# Autodesk Inventor assembly: Assembly Rotation mechanism
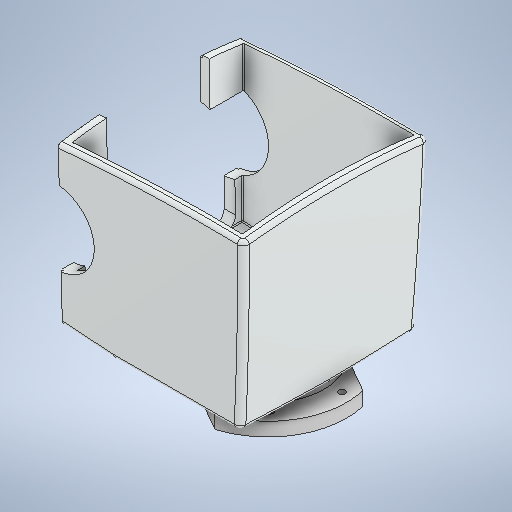
[picture p0: Inventor's stored thumbnail of the model, 512x512]
Saved by Autodesk Inventor 2025.2 (Build 292293000, 293)
## iProperties
Created: 2025-01-03
Part Number: Assembly Rotation mechanism
Document SubType Name: Assembly
Designer: marco.benkert
Author: marco.benkert
## Documents named in this file (6)
- O:\Inventor SanaBike Series\SanaBike 500 Modifield\Rotation Mechanism\Assembly Rotation mechanism.iam
- O:\Inventor SanaBike Series\SanaBike 500 Modifield\Rotation Mechanism\27-30-400 Bearing, Housing Measuring Head.ipt
- O:\Inventor SanaBike Series\SanaBike 500 Modifield\Rotation Mechanism\35-30-xxx Plain Bearing Socket.ipt
- O:\Inventor SanaBike Series\SanaBike 500 Modifield\Rotation Mechanism\25-30-100  Handlebar Cover.ipt
- O:\Inventor SanaBike Series\SanaBike 500 Modifield\Rotation Mechanism\Passscheibe 40x50x1,2 - DIN 988 (ArtNr. 42-03-007)\Passscheibe 40x50x1,2 - DIN 988 (ArtNr. 42-03-007).ipt
- O:\Inventor SanaBike Series\SanaBike 500 Modifield\Rotation Mechanism\Linsenflanschkopf (ecosyn-fix) M4x8 BN4825 (40-08-015)\Linsenflanschkopf (ecosyn-fix) M4x8 BN4825 (40-08-015).ipt
## Components (8 placed, 5 different names)
1. 27-30-400 Bearing, Housing Measuring Head:1 — Mate:6, Flush:1, Mate:7, Mate:10, Flush:2
2. 35-30-xxx Plain Bearing Socket:1 — Rotational:1, Mate:6, Flush:1
3. 25-30-100  Handlebar Cover:1 — Rotational:1, Mate:8, Mate:9, Mate:11, Mate:12, Mate:14, Mate:16
4. Passscheibe 40x50x1,2 - DIN 988 (ArtNr. 42-03-007):1 — Mate:7, Mate:8, Mate:13, Mate:15, Mate:17
5. Linsenflanschkopf (ecosyn-fix) M4x8 BN4825 (40-08-015):1 — Mate:12, Mate:13
6. Linsenflanschkopf (ecosyn-fix) M4x8 BN4825 (40-08-015):2 — Mate:16, Mate:17
7. Linsenflanschkopf (ecosyn-fix) M4x8 BN4825 (40-08-015):3 — Mate:14, Mate:15
8. Passscheibe 40x50x1,2 - DIN 988 (ArtNr. 42-03-007):2 — Mate:9, Mate:10
## Relationships (15: Mate 12, Flush 2, RevoluteJoint 1)
- Rotational:1 [RevoluteJoint]: 35-30-xxx Plain Bearing Socket:1 ↔ 25-30-100  Handlebar Cover:1
- Mate:6: 27-30-400 Bearing, Housing Measuring Head:1 ↔ 35-30-xxx Plain Bearing Socket:1
- Flush:1: 27-30-400 Bearing, Housing Measuring Head:1 ↔ 35-30-xxx Plain Bearing Socket:1
- Mate:7: 27-30-400 Bearing, Housing Measuring Head:1 ↔ Passscheibe 40x50x1,2 - DIN 988 (ArtNr. 42-03-007):1
- Mate:8: 25-30-100  Handlebar Cover:1 ↔ Passscheibe 40x50x1,2 - DIN 988 (ArtNr. 42-03-007):1
- Mate:9: 25-30-100  Handlebar Cover:1 ↔ Passscheibe 40x50x1,2 - DIN 988 (ArtNr. 42-03-007):2
- Mate:10: 27-30-400 Bearing, Housing Measuring Head:1 ↔ Passscheibe 40x50x1,2 - DIN 988 (ArtNr. 42-03-007):2
- Flush:2: 27-30-400 Bearing, Housing Measuring Head:1
- Mate:11: 25-30-100  Handlebar Cover:1
- Mate:12: 25-30-100  Handlebar Cover:1 ↔ Linsenflanschkopf (ecosyn-fix) M4x8 BN4825 (40-08-015):1
- Mate:13: Passscheibe 40x50x1,2 - DIN 988 (ArtNr. 42-03-007):1 ↔ Linsenflanschkopf (ecosyn-fix) M4x8 BN4825 (40-08-015):1
- Mate:14: 25-30-100  Handlebar Cover:1 ↔ Linsenflanschkopf (ecosyn-fix) M4x8 BN4825 (40-08-015):3
- Mate:15: Passscheibe 40x50x1,2 - DIN 988 (ArtNr. 42-03-007):1 ↔ Linsenflanschkopf (ecosyn-fix) M4x8 BN4825 (40-08-015):3
- Mate:16: 25-30-100  Handlebar Cover:1 ↔ Linsenflanschkopf (ecosyn-fix) M4x8 BN4825 (40-08-015):2
- Mate:17: Passscheibe 40x50x1,2 - DIN 988 (ArtNr. 42-03-007):1 ↔ Linsenflanschkopf (ecosyn-fix) M4x8 BN4825 (40-08-015):2
